# Autodesk Inventor assembly: leg_ass_1
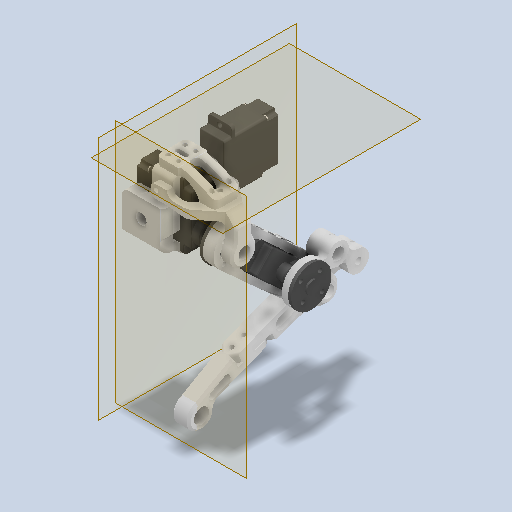
[picture p0: Inventor's stored thumbnail of the model, 512x512]
Saved by Autodesk Inventor 2022.1 (Build 261234020, 234B)
## iProperties
Created: 2019-09-26
Part Number: leg_ass_1
Document SubType Name: Assembly
Designer: kee
Mass: 55.2074 g
Surface Area: 287.545 cm^2
Volume: 46.1036 cm^3
Density: 1.19746 g/cm^3
Author: kee
## Documents named in this file (11)
- C:\Users\logic\_workspace\Quadruped_bai_servo\hardware\inventor\quadruped_bai_servo_assembly\leg_ass_1.iam
- C:\Users\logic\_workspace\Quadruped_bai_servo\hardware\inventor\quadruped_bai_servo_assembly\Emax ES08A.ipt
- C:\Users\logic\_workspace\Quadruped_bai_servo\hardware\inventor\quadruped_bai_servo_assembly\leg_1.ipt
- C:\Users\logic\_workspace\Quadruped_bai_servo\hardware\inventor\quadruped_bai_servo_assembly\leg_2.ipt
- C:\Users\logic\_workspace\Quadruped_bai_servo\hardware\inventor\quadruped_bai_servo_assembly\leg_1_2.ipt
- C:\Users\logic\_workspace\Quadruped_bai_servo\hardware\inventor\quadruped_bai_servo_assembly\leg_link_1.ipt
- C:\Users\logic\_workspace\Quadruped_bai_servo\hardware\inventor\quadruped_bai_servo_assembly\leg_link-1.ipt
- C:\Users\logic\_workspace\Quadruped_bai_servo\hardware\inventor\quadruped_bai_servo_assembly\leg_tip.ipt
- C:\Users\logic\_workspace\Quadruped_bai_servo\hardware\inventor\quadruped_bai_servo_assembly\servo_holder_1.ipt
- C:\Users\logic\_workspace\Quadruped_bai_servo\hardware\inventor\quadruped_bai_servo_assembly\hip_joint_holder_1.ipt
- C:\Users\logic\_workspace\Quadruped_bai_servo\hardware\inventor\quadruped_bai_servo_assembly\hip_holder_2.ipt
## Components (12 placed, 10 different names)
1. Emax ES08A:1 — Insert:9, Insert:10, Rotational:1
2. leg_1:1 — Insert:4, Insert:6, Insert:9, Insert:10, Insert:11, Insert:12
3. Emax ES08A:2 — Insert:14, Insert:15
4. leg_2:1 — Insert:5, Insert:6, Insert:7, Mate:2, Insert:13
5. leg_1_2:1 — Mate:2, Insert:11, Insert:12
6. leg_link_1:1 — Insert:8, Rotational:1
7. leg_link-1:1 — Insert:7, Insert:8
8. leg_tip:1 — Insert:5, Insert:13
9. servo_holder_1:1 — Insert:1, Mate:1, Insert:14, Insert:15, Insert:16, Insert:17, Flush:2, Mate:3
10. Emax ES08A:3 — Insert:16, Insert:17
11. hip_joint_holder_1:1 — Insert:2, Insert:3, Mate:1, Insert:4
12. hip_holder_2:1 — Insert:1, Insert:2, Insert:3, Flush:1
## Relationships (23: Insert 17, Mate 3, Flush 2, RevoluteJoint 1)
- Insert:1: servo_holder_1:1 ↔ hip_holder_2:1
- Insert:2: hip_joint_holder_1:1 ↔ hip_holder_2:1
- Insert:3: hip_joint_holder_1:1 ↔ hip_holder_2:1
- Mate:1: servo_holder_1:1 ↔ hip_joint_holder_1:1
- Insert:4: leg_1:1 ↔ hip_joint_holder_1:1
- Insert:5: leg_2:1 ↔ leg_tip:1
- Insert:6: leg_1:1 ↔ leg_2:1
- Insert:7: leg_2:1 ↔ leg_link-1:1
- Insert:8: leg_link_1:1 ↔ leg_link-1:1
- Mate:2: leg_2:1 ↔ leg_1_2:1
- Insert:9: Emax ES08A:1 ↔ leg_1:1
- Insert:10: Emax ES08A:1 ↔ leg_1:1
- Insert:11: leg_1:1 ↔ leg_1_2:1
- Insert:12: leg_1:1 ↔ leg_1_2:1
- Insert:13: leg_2:1 ↔ leg_tip:1
- Rotational:1 [RevoluteJoint]: Emax ES08A:1 ↔ leg_link_1:1
- Insert:14: Emax ES08A:2 ↔ servo_holder_1:1
- Insert:15: Emax ES08A:2 ↔ servo_holder_1:1
- Insert:16: servo_holder_1:1 ↔ Emax ES08A:3
- Insert:17: servo_holder_1:1 ↔ Emax ES08A:3
- Flush:1: hip_holder_2:1
- Flush:2: servo_holder_1:1
- Mate:3: servo_holder_1:1
